# Autodesk Inventor assembly: pinch_wheel
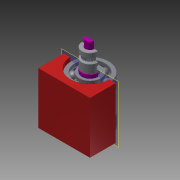
[picture p0: Inventor's stored thumbnail of the model, 180x180]
Saved by Autodesk Inventor 2014 (Build 180170000, 170)
## iProperties
Created: 2014-01-12
Part Number: pinch_wheel
Document SubType Name: Assembly
Designer: caleb
Author: caleb
## Documents named in this file (5)
- C:\cygwin\home\caleb\caleb-typea-settings\designs\pinch-wheel\pinch_wheel.iam
- C:\cygwin\home\caleb\caleb-typea-settings\designs\pinch-wheel\pinch_wheel_hobbing_jig.ipt
- C:\cygwin\home\caleb\caleb-typea-settings\designs\pinch-wheel\hobbing_jig_shaft.ipt
- C:\Documents and Settings\caleb\My Documents\Inventor\Content Center Files\R2014\en-US\DIN BEARING(1)\DIN 625 SKF - SKF 608.ipt
- C:\cygwin\home\caleb\caleb-typea-settings\designs\pinch-wheel\pinch wheel.ipt
## Components (5 placed, 4 different names)
1. pinch_wheel_hobbing_jig:1 — Mate:1, Mate:3, Mate:4, Flush:1
2. hobbing_jig_shaft:1 — Mate:5, Mate:6, Mate:7, Mate:8
3. DIN 625 SKF 608:1 — Mate:1, Mate:2, Mate:4
4. DIN 625 SKF 608:2 — Mate:2, Mate:3, Mate:5, Mate:6
5. pinch wheel:1 — Mate:7, Mate:8
## Relationships (9: Mate 8, Flush 1)
- Mate:1: pinch_wheel_hobbing_jig:1 ↔ DIN 625 SKF 608:1
- Mate:2: DIN 625 SKF 608:1 ↔ DIN 625 SKF 608:2
- Mate:3: pinch_wheel_hobbing_jig:1 ↔ DIN 625 SKF 608:2
- Mate:4: pinch_wheel_hobbing_jig:1 ↔ DIN 625 SKF 608:1
- Mate:5: hobbing_jig_shaft:1 ↔ DIN 625 SKF 608:2
- Mate:6: hobbing_jig_shaft:1 ↔ DIN 625 SKF 608:2
- Mate:7: hobbing_jig_shaft:1 ↔ pinch wheel:1
- Mate:8: hobbing_jig_shaft:1 ↔ pinch wheel:1
- Flush:1: pinch_wheel_hobbing_jig:1
